# Autodesk Inventor assembly: ASSEMBLY_Main
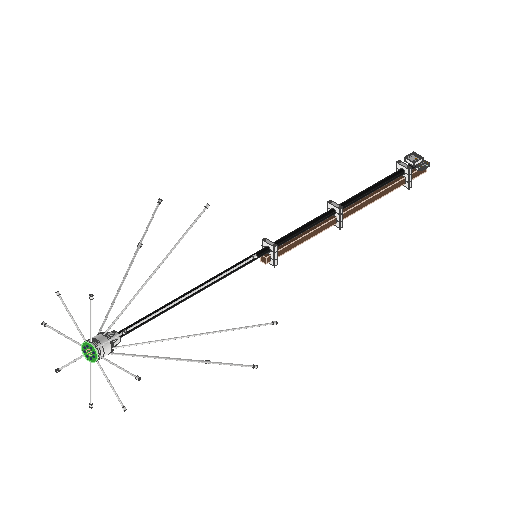
[picture p0: Inventor's stored thumbnail of the model, 512x512]
Saved by Autodesk Inventor 2026.1 (Build 301233000, 233)
## iProperties
Created: 2025-06-17
Part Number: ASSEMBLY_Main
Document SubType Name: Assembly
Designer: User
Author: User
## Documents named in this file (23)
- C:\Users\Andrzej\OneDrive\_DRIVE_SYNCH_FILES\__ BYTECHLAB PROJECTS\RF - Mostly 3D Printed Discone Antenna\MCAD\15_DISCONE_V4_KICAD\ASSEMBLY_MAIN_REVA\ASSEMBLY_Main.iam
- C:\Users\Andrzej\OneDrive\_DRIVE_SYNCH_FILES\__ BYTECHLAB PROJECTS\RF - Mostly 3D Printed Discone Antenna\MCAD\15_DISCONE_V4_KICAD\ASSEMBLY_MAIN_REVA\3DP_ASA_Top_Disc_Bottom_Half.ipt
- C:\Users\Andrzej\OneDrive\_DRIVE_SYNCH_FILES\__ BYTECHLAB PROJECTS\RF - Mostly 3D Printed Discone Antenna\MCAD\15_DISCONE_V4_KICAD\ASSEMBLY_MAIN_REVA\ASSEMBLY_Top_Disc_Rod.iam
- C:\Users\Andrzej\OneDrive\_DRIVE_SYNCH_FILES\__ BYTECHLAB PROJECTS\RF - Mostly 3D Printed Discone Antenna\MCAD\15_DISCONE_V4_KICAD\ASSEMBLY_MAIN_REVA\3DP_ASA_Top_Disc_Top_Half.ipt
- C:\Users\Andrzej\OneDrive\_DRIVE_SYNCH_FILES\__ BYTECHLAB PROJECTS\RF - Mostly 3D Printed Discone Antenna\MCAD\15_DISCONE_V4_KICAD\ASSEMBLY_MAIN_REVA\CUT_FR4_Top_Disc_PCB.ipt
- C:\Users\Andrzej\OneDrive\_DRIVE_SYNCH_FILES\__ BYTECHLAB PROJECTS\RF - Mostly 3D Printed Discone Antenna\MCAD\15_DISCONE_V4_KICAD\ASSEMBLY_MAIN_REVA\3DP_ASA_Bottom_Cone_Bottom_Half.ipt
- C:\Users\Andrzej\OneDrive\_DRIVE_SYNCH_FILES\__ BYTECHLAB PROJECTS\RF - Mostly 3D Printed Discone Antenna\MCAD\15_DISCONE_V4_KICAD\ASSEMBLY_MAIN_REVA\3DP_ASA_Bottom_Cone_Top_Half.ipt
- C:\Users\Andrzej\OneDrive\_DRIVE_SYNCH_FILES\__ BYTECHLAB PROJECTS\RF - Mostly 3D Printed Discone Antenna\MCAD\15_DISCONE_V4_KICAD\ASSEMBLY_MAIN_REVA\ASSEMBLY_Bottom_Cone_Rod.iam
- C:\Users\Andrzej\OneDrive\_DRIVE_SYNCH_FILES\__ BYTECHLAB PROJECTS\RF - Mostly 3D Printed Discone Antenna\MCAD\15_DISCONE_V4_KICAD\ASSEMBLY_MAIN_REVA\CUT_FR4_Bottom_Cone_PCB.ipt
- C:\Users\Andrzej\OneDrive\_DRIVE_SYNCH_FILES\__ BYTECHLAB PROJECTS\RF - Mostly 3D Printed Discone Antenna\MCAD\15_DISCONE_V4_KICAD\__COTS_PARTS\COTS_CarbonCenter_Fiberglass_30x28x2000mm_Pipe.ipt
- C:\Users\Andrzej\OneDrive\_DRIVE_SYNCH_FILES\__ BYTECHLAB PROJECTS\RF - Mostly 3D Printed Discone Antenna\MCAD\15_DISCONE_V4_KICAD\ASSEMBLY_MAIN_REVA\3DP_ASA_Mast_Mount.ipt
- C:\Users\Andrzej\OneDrive\_DRIVE_SYNCH_FILES\__ BYTECHLAB PROJECTS\RF - Mostly 3D Printed Discone Antenna\MCAD\15_DISCONE_V4_KICAD\ASSEMBLY_MAIN_REVA\3DP_ASA_Cone_and_Disc_Mount.ipt
- C:\Users\Andrzej\OneDrive\_DRIVE_SYNCH_FILES\__ BYTECHLAB PROJECTS\RF - Mostly 3D Printed Discone Antenna\MCAD\15_DISCONE_V4_KICAD\__COTS_PARTS\COTS_Pasternack_RG58CU_Coax_Cable\COTS_Pasternack_RG58CU_Coax_Cable.iam
- C:\Users\Andrzej\OneDrive\_DRIVE_SYNCH_FILES\__ BYTECHLAB PROJECTS\RF - Mostly 3D Printed Discone Antenna\MCAD\15_DISCONE_V4_KICAD\__CONTENT_CENTER_PARTS\en-US\DIN 934\DIN 934 - M5 x 0,8.ipt
- C:\Users\Andrzej\OneDrive\_DRIVE_SYNCH_FILES\__ BYTECHLAB PROJECTS\RF - Mostly 3D Printed Discone Antenna\MCAD\15_DISCONE_V4_KICAD\__CONTENT_CENTER_PARTS\en-US\DIN 125-1  A\DIN 125 - A 5,3.ipt
- C:\Users\Andrzej\OneDrive\_DRIVE_SYNCH_FILES\__ BYTECHLAB PROJECTS\RF - Mostly 3D Printed Discone Antenna\MCAD\15_DISCONE_V4_KICAD\__COTS_PARTS\COTS_GENERIC_DIN 912 - M5x80.ipt
- C:\Users\Andrzej\OneDrive\_DRIVE_SYNCH_FILES\__ BYTECHLAB PROJECTS\RF - Mostly 3D Printed Discone Antenna\MCAD\15_DISCONE_V4_KICAD\__COTS_PARTS\COTS_Dremec_8G206M5X40_M5x40_Nylon_Screw.ipt
- C:\Users\Andrzej\OneDrive\_DRIVE_SYNCH_FILES\__ BYTECHLAB PROJECTS\RF - Mostly 3D Printed Discone Antenna\MCAD\15_DISCONE_V4_KICAD\__COTS_PARTS\COTS_GENERIC_DIN 912 - M5x60.ipt
- C:\Users\Andrzej\OneDrive\_DRIVE_SYNCH_FILES\__ BYTECHLAB PROJECTS\RF - Mostly 3D Printed Discone Antenna\MCAD\15_DISCONE_V4_KICAD\ASSEMBLY_MAIN_REVA\ASSEMBLY_Balcony_Mounting_Clamp.iam
- C:\Users\Andrzej\OneDrive\_DRIVE_SYNCH_FILES\__ BYTECHLAB PROJECTS\RF - Mostly 3D Printed Discone Antenna\MCAD\15_DISCONE_V4_KICAD\__COTS_PARTS\COTS_GENERIC_Balcony_Railing.ipt
- C:\Users\Andrzej\OneDrive\_DRIVE_SYNCH_FILES\__ BYTECHLAB PROJECTS\RF - Mostly 3D Printed Discone Antenna\MCAD\15_DISCONE_V4_KICAD\ASSEMBLY_PREAMP_REVA\ASSEMBLY_Preamp.iam
- C:\Users\Andrzej\OneDrive\_DRIVE_SYNCH_FILES\__ BYTECHLAB PROJECTS\RF - Mostly 3D Printed Discone Antenna\MCAD\15_DISCONE_V4_KICAD\ASSEMBLY_BIAS_TEE_REVA\ASSEMBLY_Bias_Tee.iam
- C:\Users\Andrzej\OneDrive\_DRIVE_SYNCH_FILES\__ BYTECHLAB PROJECTS\RF - Mostly 3D Printed Discone Antenna\MCAD\15_DISCONE_V4_KICAD\__COTS_PARTS\COTS_BOSSARD_B5_BN81_M5_Nylon_Nuts.ipt
## Components (76 placed, 22 different names)
1. 3DP_ASA_Top_Disc_Bottom_Half:1 — Mate:1, Mate:2, Mate:3, Mate:4, Angle:1, Mate:5, Mate:6, Mate:7, Mate:11, Mate:27
2. 3DP_ASA_Top_Disc_Top_Half:1 — Mate:5, Mate:6, Mate:7, Mate:8, Mate:9, Mate:10, Mate:26, Mate:64, Mate:65, Mate:66, Mate:67, Mate:68, Mate:69, Mate:70, Mate:71
3. CUT_FR4_Top_Disc_PCB:1 — Mate:8, Mate:9, Mate:10, Mate:72, Mate:73, Mate:74, Mate:75, Mate:76, Mate:77, Mate:78, Mate:79
4. 3DP_ASA_Bottom_Cone_Bottom_Half:1 — Mate:11, Mate:13, Mate:14, Flush:1, Mate:15, Mate:16, Angle:2, Mate:19, Mate:20, Mate:22, Mate:30, Mate:36
5. 3DP_ASA_Bottom_Cone_Top_Half:1 — Mate:13, Mate:14, Flush:1, Flush:2, Mate:17, Mate:18, Mate:23, Mate:24, Mate:25
6. CUT_FR4_Bottom_Cone_PCB:1 — Flush:2, Mate:17, Tangent:1, Mate:31
7. COTS_CarbonCenter_Fiberglass_30x28x2000mm_Pipe:1 — Mate:18, Mate:19, Mate:21, Mate:29, Mate:82, Mate:83, Mate:84, Flush:3, Mate:89, Flush:4
8. 3DP_ASA_Mast_Mount:1 — Mate:20, Mate:21, Mate:22, Mate:29, Insert:9, Insert:10, Insert:11, Insert:12, Insert:13, Insert:14, Insert:15, Insert:16, Mate:32, Mate:34, Mate:35, Mate:37, Mate:38, Mate:39, Mate:40, Insert:17, Insert:18, Mate:80
9. 3DP_ASA_Cone_and_Disc_Mount:1 — Mate:23, Mate:24, Mate:25, Mate:26, Mate:27, Insert:1, Insert:2, Insert:3, Insert:4, Insert:5, Insert:6, Insert:7, Insert:8, Angle:3, Angle:4, Angle:5, Angle:6, Angle:7, Angle:8, Angle:9, Angle:10, Mate:48, Mate:49, Mate:50, Mate:51, Mate:52, Mate:53, Mate:54, Mate:55, Mate:56, Mate:57, Mate:58, Mate:59, Mate:60, Mate:61, Mate:62, Mate:63, Angle:11, Angle:12, Angle:13, Angle:14, Angle:15, Angle:16, Angle:17, Angle:18
10. COTS_Pasternack_RG58CU_Coax_Cable:1 [sub-assembly] — Mate:30, Mate:31
11. ASSEMBLY_Balcony_Mounting_Clamp:1 [sub-assembly] — Mate:82, Mate:85, Angle:20, Angle:21, Flush:3, Mate:86, Angle:22
12. ASSEMBLY_Balcony_Mounting_Clamp:2 [sub-assembly] — Mate:83, Angle:19, Angle:20, Mate:86, Mate:87
13. ASSEMBLY_Balcony_Mounting_Clamp:3 [sub-assembly] — Mate:84, Mate:85, Angle:19, Mate:88
14. COTS_GENERIC_Balcony_Railing:1 — Mate:87, Mate:88
15. ASSEMBLY_Preamp:1 [sub-assembly] — Mate:89, Angle:22, Flush:4, Flush:5, Flush:6, Mate:90
16. ASSEMBLY_Bias_Tee:1 [sub-assembly] — Flush:5, Flush:6, Mate:90
17. DIN 934 - replaced by DIN EN 24032/28673/28674 M5:17 — Insert:19
18. COTS_GENERIC_DIN 912 - M5x60:1 — Mate:80, Mate:81
19. DIN 125-1 A A 5,3:10 — Insert:18, Insert:19
20. DIN 125-1 A A 5,3:9 — Insert:17, Mate:81
21. COTS_Dremec_8G206M5X40_M5x40_Nylon_Screw:8 — Mate:68, Mate:75
22. COTS_Dremec_8G206M5X40_M5x40_Nylon_Screw:7 — Mate:71, Mate:78
23. COTS_Dremec_8G206M5X40_M5x40_Nylon_Screw:6 — Mate:70, Mate:77
24. COTS_Dremec_8G206M5X40_M5x40_Nylon_Screw:5 — Mate:69, Mate:76
25. COTS_Dremec_8G206M5X40_M5x40_Nylon_Screw:4 — Mate:64, Mate:79
26. COTS_Dremec_8G206M5X40_M5x40_Nylon_Screw:3 — Mate:67, Mate:74
27. COTS_Dremec_8G206M5X40_M5x40_Nylon_Screw:2 — Mate:66, Mate:72
28. COTS_Dremec_8G206M5X40_M5x40_Nylon_Screw:1 — Mate:65, Mate:73
29. COTS_BOSSARD_B5_BN81_M5_Nylon_Nuts:16 — Mate:51, Mate:57, Angle:14
30. COTS_BOSSARD_B5_BN81_M5_Nylon_Nuts:17 — Mate:54, Mate:60, Angle:17
31. COTS_BOSSARD_B5_BN81_M5_Nylon_Nuts:18 — Mate:55, Mate:59, Angle:16
32. COTS_BOSSARD_B5_BN81_M5_Nylon_Nuts:19 — Mate:52, Mate:58, Angle:15
33. COTS_BOSSARD_B5_BN81_M5_Nylon_Nuts:20 — Mate:48, Mate:62, Angle:11
34. COTS_BOSSARD_B5_BN81_M5_Nylon_Nuts:21 — Mate:49, Mate:63, Angle:12
35. COTS_BOSSARD_B5_BN81_M5_Nylon_Nuts:22 — Mate:50, Mate:56, Angle:13
36. COTS_BOSSARD_B5_BN81_M5_Nylon_Nuts:23 — Mate:53, Mate:61, Angle:18
37. DIN 934 - replaced by DIN EN 24032/28673/28674 M5:1 — Insert:1, Angle:5
38. DIN 934 - replaced by DIN EN 24032/28673/28674 M5:2 — Insert:2, Angle:7
39. DIN 934 - replaced by DIN EN 24032/28673/28674 M5:3 — Insert:3, Angle:3
40. DIN 934 - replaced by DIN EN 24032/28673/28674 M5:4 — Insert:4, Angle:4
41. DIN 934 - replaced by DIN EN 24032/28673/28674 M5:5 — Insert:5, Angle:8
42. DIN 934 - replaced by DIN EN 24032/28673/28674 M5:6 — Insert:6, Angle:6
43. DIN 934 - replaced by DIN EN 24032/28673/28674 M5:7 — Insert:7, Angle:9
44. DIN 934 - replaced by DIN EN 24032/28673/28674 M5:8 — Insert:8, Angle:10
45. DIN 125-1 A A 5,3:1 — Insert:9, Mate:41
46. DIN 125-1 A A 5,3:2 — Insert:10, Mate:46
47. DIN 125-1 A A 5,3:3 — Insert:11, Mate:42
48. DIN 125-1 A A 5,3:4 — Insert:12, Mate:47
49. DIN 125-1 A A 5,3:5 — Insert:13, Mate:43
50. DIN 125-1 A A 5,3:6 — Insert:14, Mate:45
51. DIN 125-1 A A 5,3:7 — Insert:15, Mate:33
52. DIN 125-1 A A 5,3:8 — Insert:16, Mate:44
53. COTS_GENERIC_DIN 912 - M5x80:1 — Mate:32, Mate:33
54. COTS_GENERIC_DIN 912 - M5x80:2 — Mate:34, Mate:47
55. COTS_GENERIC_DIN 912 - M5x80:3 — Mate:35, Mate:46
56. COTS_GENERIC_DIN 912 - M5x80:4 — Mate:36, Mate:45
57. COTS_GENERIC_DIN 912 - M5x80:5 — Mate:38, Mate:43
58. COTS_GENERIC_DIN 912 - M5x80:6 — Mate:39, Mate:42
59. COTS_GENERIC_DIN 912 - M5x80:7 — Mate:40, Mate:41
60. COTS_GENERIC_DIN 912 - M5x80:8 — Mate:37, Mate:44
61. ASSEMBLY_Top_Disc_Rod:1 [sub-assembly] — Mate:3, Mate:4, Angle:1
62. ASSEMBLY_Top_Disc_Rod:2 [sub-assembly]
63. ASSEMBLY_Top_Disc_Rod:3 [sub-assembly]
64. ASSEMBLY_Top_Disc_Rod:4 [sub-assembly] — Mate:28
65. ASSEMBLY_Top_Disc_Rod:5 [sub-assembly]
66. ASSEMBLY_Top_Disc_Rod:6 [sub-assembly]
67. ASSEMBLY_Top_Disc_Rod:7 [sub-assembly]
68. ASSEMBLY_Top_Disc_Rod:8 [sub-assembly]
69. ASSEMBLY_Bottom_Cone_Rod:1 [sub-assembly] — Mate:15, Mate:16, Angle:2
70. ASSEMBLY_Bottom_Cone_Rod:2 [sub-assembly]
71. ASSEMBLY_Bottom_Cone_Rod:3 [sub-assembly]
72. ASSEMBLY_Bottom_Cone_Rod:4 [sub-assembly]
73. ASSEMBLY_Bottom_Cone_Rod:5 [sub-assembly]
74. ASSEMBLY_Bottom_Cone_Rod:6 [sub-assembly]
75. ASSEMBLY_Bottom_Cone_Rod:7 [sub-assembly] — Tangent:1
76. ASSEMBLY_Bottom_Cone_Rod:8 [sub-assembly]
## Component patterns: (8 elements, first: ASSEMBLY_Top_Disc_Rod:1), (8 elements, first: ASSEMBLY_Bottom_Cone_Rod:1)
## Relationships (137: Mate 89, Angle 22, Insert 19, Flush 6, Tangent 1)
- Mate:1: 3DP_ASA_Top_Disc_Bottom_Half:1
- Mate:2: 3DP_ASA_Top_Disc_Bottom_Half:1
- Mate:3: 3DP_ASA_Top_Disc_Bottom_Half:1 ↔ ASSEMBLY_Top_Disc_Rod:1
- Mate:4 (16 mm): 3DP_ASA_Top_Disc_Bottom_Half:1 ↔ ASSEMBLY_Top_Disc_Rod:1
- Angle:1 (-90 deg): 3DP_ASA_Top_Disc_Bottom_Half:1 ↔ ASSEMBLY_Top_Disc_Rod:1
- Mate:5 (0.5 mm): 3DP_ASA_Top_Disc_Bottom_Half:1 ↔ 3DP_ASA_Top_Disc_Top_Half:1
- Mate:6: 3DP_ASA_Top_Disc_Bottom_Half:1 ↔ 3DP_ASA_Top_Disc_Top_Half:1
- Mate:7: 3DP_ASA_Top_Disc_Bottom_Half:1 ↔ 3DP_ASA_Top_Disc_Top_Half:1
- Mate:8: 3DP_ASA_Top_Disc_Top_Half:1 ↔ CUT_FR4_Top_Disc_PCB:1
- Mate:9: 3DP_ASA_Top_Disc_Top_Half:1 ↔ CUT_FR4_Top_Disc_PCB:1
- Mate:10: 3DP_ASA_Top_Disc_Top_Half:1 ↔ CUT_FR4_Top_Disc_PCB:1
- Mate:11: 3DP_ASA_Top_Disc_Bottom_Half:1 ↔ 3DP_ASA_Bottom_Cone_Bottom_Half:1
- Mate:13: 3DP_ASA_Bottom_Cone_Bottom_Half:1 ↔ 3DP_ASA_Bottom_Cone_Top_Half:1
- Mate:14: 3DP_ASA_Bottom_Cone_Bottom_Half:1 ↔ 3DP_ASA_Bottom_Cone_Top_Half:1
- Flush:1 (11 mm): 3DP_ASA_Bottom_Cone_Bottom_Half:1 ↔ 3DP_ASA_Bottom_Cone_Top_Half:1
- Mate:15: 3DP_ASA_Bottom_Cone_Bottom_Half:1 ↔ ASSEMBLY_Bottom_Cone_Rod:1
- Mate:16 (3 mm): 3DP_ASA_Bottom_Cone_Bottom_Half:1 ↔ ASSEMBLY_Bottom_Cone_Rod:1
- Angle:2 (0 deg): 3DP_ASA_Bottom_Cone_Bottom_Half:1 ↔ ASSEMBLY_Bottom_Cone_Rod:1
- Flush:2 (1 mm): 3DP_ASA_Bottom_Cone_Top_Half:1 ↔ CUT_FR4_Bottom_Cone_PCB:1
- Mate:17: 3DP_ASA_Bottom_Cone_Top_Half:1 ↔ CUT_FR4_Bottom_Cone_PCB:1
- Tangent:1 (-0.2 mm): CUT_FR4_Bottom_Cone_PCB:1 ↔ ASSEMBLY_Bottom_Cone_Rod:7
- Mate:18: 3DP_ASA_Bottom_Cone_Top_Half:1 ↔ COTS_CarbonCenter_Fiberglass_30x28x2000mm_Pipe:1
- Mate:19: 3DP_ASA_Bottom_Cone_Bottom_Half:1 ↔ COTS_CarbonCenter_Fiberglass_30x28x2000mm_Pipe:1
- Mate:20: 3DP_ASA_Bottom_Cone_Bottom_Half:1 ↔ 3DP_ASA_Mast_Mount:1
- Mate:21: COTS_CarbonCenter_Fiberglass_30x28x2000mm_Pipe:1 ↔ 3DP_ASA_Mast_Mount:1
- Mate:22: 3DP_ASA_Bottom_Cone_Bottom_Half:1 ↔ 3DP_ASA_Mast_Mount:1
- Mate:23: 3DP_ASA_Bottom_Cone_Top_Half:1 ↔ 3DP_ASA_Cone_and_Disc_Mount:1
- Mate:24: 3DP_ASA_Bottom_Cone_Top_Half:1 ↔ 3DP_ASA_Cone_and_Disc_Mount:1
- Mate:25: 3DP_ASA_Bottom_Cone_Top_Half:1 ↔ 3DP_ASA_Cone_and_Disc_Mount:1
- Mate:26: 3DP_ASA_Top_Disc_Top_Half:1 ↔ 3DP_ASA_Cone_and_Disc_Mount:1
- Mate:27: 3DP_ASA_Top_Disc_Bottom_Half:1 ↔ 3DP_ASA_Cone_and_Disc_Mount:1
- Mate:28: ASSEMBLY_Top_Disc_Rod:4
- Mate:29: COTS_CarbonCenter_Fiberglass_30x28x2000mm_Pipe:1 ↔ 3DP_ASA_Mast_Mount:1
- Mate:30: 3DP_ASA_Bottom_Cone_Bottom_Half:1 ↔ COTS_Pasternack_RG58CU_Coax_Cable:1
- Mate:31: CUT_FR4_Bottom_Cone_PCB:1 ↔ COTS_Pasternack_RG58CU_Coax_Cable:1
- Insert:1: 3DP_ASA_Cone_and_Disc_Mount:1 ↔ DIN 934 - replaced by DIN EN 24032/28673/28674 M5:1
- Insert:2: 3DP_ASA_Cone_and_Disc_Mount:1 ↔ DIN 934 - replaced by DIN EN 24032/28673/28674 M5:2
- Insert:3: 3DP_ASA_Cone_and_Disc_Mount:1 ↔ DIN 934 - replaced by DIN EN 24032/28673/28674 M5:3
- Insert:4: 3DP_ASA_Cone_and_Disc_Mount:1 ↔ DIN 934 - replaced by DIN EN 24032/28673/28674 M5:4
- Insert:5: 3DP_ASA_Cone_and_Disc_Mount:1 ↔ DIN 934 - replaced by DIN EN 24032/28673/28674 M5:5
- Insert:6: 3DP_ASA_Cone_and_Disc_Mount:1 ↔ DIN 934 - replaced by DIN EN 24032/28673/28674 M5:6
- Insert:7: 3DP_ASA_Cone_and_Disc_Mount:1 ↔ DIN 934 - replaced by DIN EN 24032/28673/28674 M5:7
- Insert:8: 3DP_ASA_Cone_and_Disc_Mount:1 ↔ DIN 934 - replaced by DIN EN 24032/28673/28674 M5:8
- Angle:3 (0 deg): 3DP_ASA_Cone_and_Disc_Mount:1 ↔ DIN 934 - replaced by DIN EN 24032/28673/28674 M5:3
- Angle:4 (0 deg): 3DP_ASA_Cone_and_Disc_Mount:1 ↔ DIN 934 - replaced by DIN EN 24032/28673/28674 M5:4
- Angle:5 (0 deg): 3DP_ASA_Cone_and_Disc_Mount:1 ↔ DIN 934 - replaced by DIN EN 24032/28673/28674 M5:1
- Angle:6 (0 deg): 3DP_ASA_Cone_and_Disc_Mount:1 ↔ DIN 934 - replaced by DIN EN 24032/28673/28674 M5:6
- Angle:7 (0 deg): 3DP_ASA_Cone_and_Disc_Mount:1 ↔ DIN 934 - replaced by DIN EN 24032/28673/28674 M5:2
- Angle:8 (0 deg): 3DP_ASA_Cone_and_Disc_Mount:1 ↔ DIN 934 - replaced by DIN EN 24032/28673/28674 M5:5
- Angle:9 (0 deg): 3DP_ASA_Cone_and_Disc_Mount:1 ↔ DIN 934 - replaced by DIN EN 24032/28673/28674 M5:7
- Angle:10 (0 deg): 3DP_ASA_Cone_and_Disc_Mount:1 ↔ DIN 934 - replaced by DIN EN 24032/28673/28674 M5:8
- Insert:9: 3DP_ASA_Mast_Mount:1 ↔ DIN 125-1 A A 5,3:1
- Insert:10: 3DP_ASA_Mast_Mount:1 ↔ DIN 125-1 A A 5,3:2
- Insert:11: 3DP_ASA_Mast_Mount:1 ↔ DIN 125-1 A A 5,3:3
- Insert:12: 3DP_ASA_Mast_Mount:1 ↔ DIN 125-1 A A 5,3:4
- Insert:13: 3DP_ASA_Mast_Mount:1 ↔ DIN 125-1 A A 5,3:5
- Insert:14: 3DP_ASA_Mast_Mount:1 ↔ DIN 125-1 A A 5,3:6
- Insert:15: 3DP_ASA_Mast_Mount:1 ↔ DIN 125-1 A A 5,3:7
- Insert:16: 3DP_ASA_Mast_Mount:1 ↔ DIN 125-1 A A 5,3:8
- Mate:32: 3DP_ASA_Mast_Mount:1 ↔ COTS_GENERIC_DIN 912 - M5x80:1
- Mate:33: DIN 125-1 A A 5,3:7 ↔ COTS_GENERIC_DIN 912 - M5x80:1
- Mate:34: 3DP_ASA_Mast_Mount:1 ↔ COTS_GENERIC_DIN 912 - M5x80:2
- Mate:35: 3DP_ASA_Mast_Mount:1 ↔ COTS_GENERIC_DIN 912 - M5x80:3
- Mate:36: 3DP_ASA_Bottom_Cone_Bottom_Half:1 ↔ COTS_GENERIC_DIN 912 - M5x80:4
- Mate:37: 3DP_ASA_Mast_Mount:1 ↔ COTS_GENERIC_DIN 912 - M5x80:8
- Mate:38: 3DP_ASA_Mast_Mount:1 ↔ COTS_GENERIC_DIN 912 - M5x80:5
- Mate:39: 3DP_ASA_Mast_Mount:1 ↔ COTS_GENERIC_DIN 912 - M5x80:6
- Mate:40: 3DP_ASA_Mast_Mount:1 ↔ COTS_GENERIC_DIN 912 - M5x80:7
- Mate:41: DIN 125-1 A A 5,3:1 ↔ COTS_GENERIC_DIN 912 - M5x80:7
- Mate:42: DIN 125-1 A A 5,3:3 ↔ COTS_GENERIC_DIN 912 - M5x80:6
- Mate:43: DIN 125-1 A A 5,3:5 ↔ COTS_GENERIC_DIN 912 - M5x80:5
- Mate:44: DIN 125-1 A A 5,3:8 ↔ COTS_GENERIC_DIN 912 - M5x80:8
- Mate:45: DIN 125-1 A A 5,3:6 ↔ COTS_GENERIC_DIN 912 - M5x80:4
- Mate:46: DIN 125-1 A A 5,3:2 ↔ COTS_GENERIC_DIN 912 - M5x80:3
- Mate:47: DIN 125-1 A A 5,3:4 ↔ COTS_GENERIC_DIN 912 - M5x80:2
- Mate:48: 3DP_ASA_Cone_and_Disc_Mount:1 ↔ COTS_BOSSARD_B5_BN81_M5_Nylon_Nuts:20
- Mate:49: 3DP_ASA_Cone_and_Disc_Mount:1 ↔ COTS_BOSSARD_B5_BN81_M5_Nylon_Nuts:21
- Mate:50: 3DP_ASA_Cone_and_Disc_Mount:1 ↔ COTS_BOSSARD_B5_BN81_M5_Nylon_Nuts:22
- Mate:51: 3DP_ASA_Cone_and_Disc_Mount:1 ↔ COTS_BOSSARD_B5_BN81_M5_Nylon_Nuts:16
- Mate:52: 3DP_ASA_Cone_and_Disc_Mount:1 ↔ COTS_BOSSARD_B5_BN81_M5_Nylon_Nuts:19
- Mate:53: 3DP_ASA_Cone_and_Disc_Mount:1 ↔ COTS_BOSSARD_B5_BN81_M5_Nylon_Nuts:23
- Mate:54: 3DP_ASA_Cone_and_Disc_Mount:1 ↔ COTS_BOSSARD_B5_BN81_M5_Nylon_Nuts:17
- Mate:55: 3DP_ASA_Cone_and_Disc_Mount:1 ↔ COTS_BOSSARD_B5_BN81_M5_Nylon_Nuts:18
- Mate:56: 3DP_ASA_Cone_and_Disc_Mount:1 ↔ COTS_BOSSARD_B5_BN81_M5_Nylon_Nuts:22
- Mate:57: 3DP_ASA_Cone_and_Disc_Mount:1 ↔ COTS_BOSSARD_B5_BN81_M5_Nylon_Nuts:16
- Mate:58: 3DP_ASA_Cone_and_Disc_Mount:1 ↔ COTS_BOSSARD_B5_BN81_M5_Nylon_Nuts:19
- Mate:59: 3DP_ASA_Cone_and_Disc_Mount:1 ↔ COTS_BOSSARD_B5_BN81_M5_Nylon_Nuts:18
- Mate:60: 3DP_ASA_Cone_and_Disc_Mount:1 ↔ COTS_BOSSARD_B5_BN81_M5_Nylon_Nuts:17
- Mate:61: 3DP_ASA_Cone_and_Disc_Mount:1 ↔ COTS_BOSSARD_B5_BN81_M5_Nylon_Nuts:23
- Mate:62: 3DP_ASA_Cone_and_Disc_Mount:1 ↔ COTS_BOSSARD_B5_BN81_M5_Nylon_Nuts:20
- Mate:63: 3DP_ASA_Cone_and_Disc_Mount:1 ↔ COTS_BOSSARD_B5_BN81_M5_Nylon_Nuts:21
- Angle:11 (0 deg): 3DP_ASA_Cone_and_Disc_Mount:1 ↔ COTS_BOSSARD_B5_BN81_M5_Nylon_Nuts:20
- Angle:12 (0 deg): 3DP_ASA_Cone_and_Disc_Mount:1 ↔ COTS_BOSSARD_B5_BN81_M5_Nylon_Nuts:21
- Angle:13 (0 deg): 3DP_ASA_Cone_and_Disc_Mount:1 ↔ COTS_BOSSARD_B5_BN81_M5_Nylon_Nuts:22
- Angle:14 (0 deg): 3DP_ASA_Cone_and_Disc_Mount:1 ↔ COTS_BOSSARD_B5_BN81_M5_Nylon_Nuts:16
- Angle:15 (0 deg): 3DP_ASA_Cone_and_Disc_Mount:1 ↔ COTS_BOSSARD_B5_BN81_M5_Nylon_Nuts:19
- Angle:16 (0 deg): 3DP_ASA_Cone_and_Disc_Mount:1 ↔ COTS_BOSSARD_B5_BN81_M5_Nylon_Nuts:18
- Angle:17 (0 deg): 3DP_ASA_Cone_and_Disc_Mount:1 ↔ COTS_BOSSARD_B5_BN81_M5_Nylon_Nuts:17
- Angle:18 (0 deg): 3DP_ASA_Cone_and_Disc_Mount:1 ↔ COTS_BOSSARD_B5_BN81_M5_Nylon_Nuts:23
- Mate:64: 3DP_ASA_Top_Disc_Top_Half:1 ↔ COTS_Dremec_8G206M5X40_M5x40_Nylon_Screw:4
- Mate:65: 3DP_ASA_Top_Disc_Top_Half:1 ↔ COTS_Dremec_8G206M5X40_M5x40_Nylon_Screw:1
- Mate:66: 3DP_ASA_Top_Disc_Top_Half:1 ↔ COTS_Dremec_8G206M5X40_M5x40_Nylon_Screw:2
- Mate:67: 3DP_ASA_Top_Disc_Top_Half:1 ↔ COTS_Dremec_8G206M5X40_M5x40_Nylon_Screw:3
- Mate:68: 3DP_ASA_Top_Disc_Top_Half:1 ↔ COTS_Dremec_8G206M5X40_M5x40_Nylon_Screw:8
- Mate:69: 3DP_ASA_Top_Disc_Top_Half:1 ↔ COTS_Dremec_8G206M5X40_M5x40_Nylon_Screw:5
- Mate:70: 3DP_ASA_Top_Disc_Top_Half:1 ↔ COTS_Dremec_8G206M5X40_M5x40_Nylon_Screw:6
- Mate:71: 3DP_ASA_Top_Disc_Top_Half:1 ↔ COTS_Dremec_8G206M5X40_M5x40_Nylon_Screw:7
- Mate:72: CUT_FR4_Top_Disc_PCB:1 ↔ COTS_Dremec_8G206M5X40_M5x40_Nylon_Screw:2
- Mate:73: CUT_FR4_Top_Disc_PCB:1 ↔ COTS_Dremec_8G206M5X40_M5x40_Nylon_Screw:1
- Mate:74: CUT_FR4_Top_Disc_PCB:1 ↔ COTS_Dremec_8G206M5X40_M5x40_Nylon_Screw:3
- Mate:75: CUT_FR4_Top_Disc_PCB:1 ↔ COTS_Dremec_8G206M5X40_M5x40_Nylon_Screw:8
- Mate:76: CUT_FR4_Top_Disc_PCB:1 ↔ COTS_Dremec_8G206M5X40_M5x40_Nylon_Screw:5
- Mate:77: CUT_FR4_Top_Disc_PCB:1 ↔ COTS_Dremec_8G206M5X40_M5x40_Nylon_Screw:6
- Mate:78: CUT_FR4_Top_Disc_PCB:1 ↔ COTS_Dremec_8G206M5X40_M5x40_Nylon_Screw:7
- Mate:79: CUT_FR4_Top_Disc_PCB:1 ↔ COTS_Dremec_8G206M5X40_M5x40_Nylon_Screw:4
- Insert:17: 3DP_ASA_Mast_Mount:1 ↔ DIN 125-1 A A 5,3:9
- Insert:18: 3DP_ASA_Mast_Mount:1 ↔ DIN 125-1 A A 5,3:10
- Mate:80: 3DP_ASA_Mast_Mount:1 ↔ COTS_GENERIC_DIN 912 - M5x60:1
- Mate:81: COTS_GENERIC_DIN 912 - M5x60:1 ↔ DIN 125-1 A A 5,3:9
- Insert:19: DIN 934 - replaced by DIN EN 24032/28673/28674 M5:17 ↔ DIN 125-1 A A 5,3:10
- Mate:82: COTS_CarbonCenter_Fiberglass_30x28x2000mm_Pipe:1 ↔ ASSEMBLY_Balcony_Mounting_Clamp:1
- Mate:83: COTS_CarbonCenter_Fiberglass_30x28x2000mm_Pipe:1 ↔ ASSEMBLY_Balcony_Mounting_Clamp:2
- Mate:84: COTS_CarbonCenter_Fiberglass_30x28x2000mm_Pipe:1 ↔ ASSEMBLY_Balcony_Mounting_Clamp:3
- Mate:85 (820 mm): ASSEMBLY_Balcony_Mounting_Clamp:1 ↔ ASSEMBLY_Balcony_Mounting_Clamp:3
- Angle:19 (0 deg): ASSEMBLY_Balcony_Mounting_Clamp:2 ↔ ASSEMBLY_Balcony_Mounting_Clamp:3
- Angle:20 (0 deg): ASSEMBLY_Balcony_Mounting_Clamp:1 ↔ ASSEMBLY_Balcony_Mounting_Clamp:2
- Angle:21 (0 deg): ASSEMBLY_Balcony_Mounting_Clamp:1
- Flush:3 (100 mm): COTS_CarbonCenter_Fiberglass_30x28x2000mm_Pipe:1 ↔ ASSEMBLY_Balcony_Mounting_Clamp:1
- Mate:86 (410 mm): ASSEMBLY_Balcony_Mounting_Clamp:1 ↔ ASSEMBLY_Balcony_Mounting_Clamp:2
- Mate:87 (0.05 mm): ASSEMBLY_Balcony_Mounting_Clamp:2 ↔ COTS_GENERIC_Balcony_Railing:1
- Mate:88 (0.05 mm): ASSEMBLY_Balcony_Mounting_Clamp:3 ↔ COTS_GENERIC_Balcony_Railing:1
- Mate:89: COTS_CarbonCenter_Fiberglass_30x28x2000mm_Pipe:1 ↔ ASSEMBLY_Preamp:1
- Angle:22 (0 deg): ASSEMBLY_Balcony_Mounting_Clamp:1 ↔ ASSEMBLY_Preamp:1
- Flush:4 (20 mm): COTS_CarbonCenter_Fiberglass_30x28x2000mm_Pipe:1 ↔ ASSEMBLY_Preamp:1
- Flush:5: ASSEMBLY_Preamp:1 ↔ ASSEMBLY_Bias_Tee:1
- Flush:6: ASSEMBLY_Preamp:1 ↔ ASSEMBLY_Bias_Tee:1
- Mate:90 (20 mm): ASSEMBLY_Preamp:1 ↔ ASSEMBLY_Bias_Tee:1
